# Autodesk Inventor assembly: outside_sleds_MIR
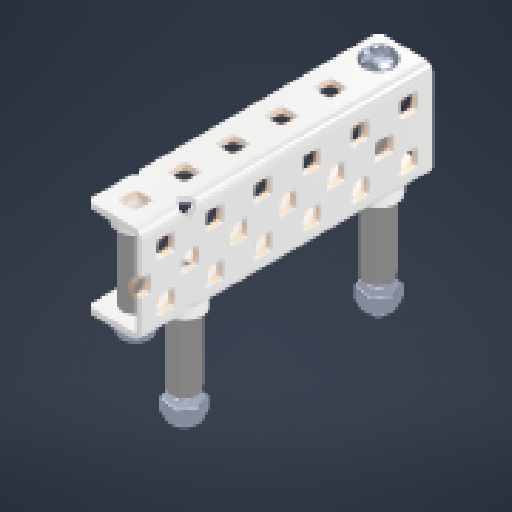
[picture p0: Inventor's stored thumbnail of the model, 512x512]
Saved by Autodesk Inventor 2023 (Build 270158000, 158)
## iProperties
Created: 2023-08-07
Part Number: outside_sleds_MIR
Document SubType Name: Assembly
Designer: srbel
Author: srbel
## Documents named in this file (10)
- C:\CAD\OverUnderCAD\Drive\outside_sleds_MIR.iam
- C:\CAD\OverUnderCAD\VEX-CAD-Inventor-1.4.0\Structure\C Channel\Aluminum 1x2x1\Alu C 1x2x1x6_MIR.ipt
- C:\CAD\OverUnderCAD\VEX-CAD-Inventor-1.4.0\Motion\Spacers\Spacer Nylon .313 OD\NSpacer .313 OD x .125.ipt
- C:\CAD\OverUnderCAD\VEX-CAD-Inventor-1.4.0\Motion\Spacers\Spacer Nylon .313 OD.ipt
- C:\CAD\OverUnderCAD\VEX-CAD-Inventor-1.4.0\Structure\Standoff\Standoff .75.ipt
- C:\CAD\OverUnderCAD\VEX-CAD-Inventor-1.4.0\Structure\Standoff.ipt
- C:\CAD\OverUnderCAD\VEX-CAD-Inventor-1.4.0\Structure\Hardware\Screw Steel - Star\SScrew Star Threaded 2.250.ipt
- C:\CAD\OverUnderCAD\VEX-CAD-Inventor-1.4.0\Structure\Hardware\Screw Steel - Star.ipt
- C:\CAD\OverUnderCAD\VEX-CAD-Inventor-1.4.0\Structure\Hardware\Screw Steel - Star\SScrew Star Threaded 1.250.ipt
- C:\CAD\OverUnderCAD\VEX-CAD-Inventor-1.4.0\Structure\Hardware\Nut Thin Nylock.ipt
## Components (14 placed, 6 different names)
1. Alu C 1x2x1x6_MIR:1 — Insert:1, Insert:3, Insert:6, Insert:7, Insert:9, Insert:11, Insert:12
2. NSpacer .313 OD x .125:1 — Insert:1, Insert:2
3. Standoff .75:1 — Insert:2
4. NSpacer .313 OD x .125:2 — Insert:3, Insert:4
5. Standoff .75:2 — Insert:4
6. NSpacer .313 OD x .125:3 — Insert:6, Insert:5
7. Standoff .75:3 — Insert:5, Insert:14
8. NSpacer .313 OD x .125:4 — Insert:7, Insert:8
9. Standoff .75:4 — Insert:8, Insert:13
10. SScrew Star Threaded 2.250:1 — Insert:9
11. SScrew Star Threaded 1.250:3 — Insert:11
12. Nut Thin Nylock:1 — Insert:12
13. Nut Thin Nylock:2 — Insert:13
14. Nut Thin Nylock:3 — Insert:14
## Relationships (13: Insert 13)
- Insert:1: Alu C 1x2x1x6_MIR:1 ↔ NSpacer .313 OD x .125:1
- Insert:2: NSpacer .313 OD x .125:1 ↔ Standoff .75:1
- Insert:3: Alu C 1x2x1x6_MIR:1 ↔ NSpacer .313 OD x .125:2
- Insert:4: NSpacer .313 OD x .125:2 ↔ Standoff .75:2
- Insert:6 (1.5875 mm): Alu C 1x2x1x6_MIR:1 ↔ NSpacer .313 OD x .125:3
- Insert:5: NSpacer .313 OD x .125:3 ↔ Standoff .75:3
- Insert:7 (1.5875 mm): Alu C 1x2x1x6_MIR:1 ↔ NSpacer .313 OD x .125:4
- Insert:8: NSpacer .313 OD x .125:4 ↔ Standoff .75:4
- Insert:9: Alu C 1x2x1x6_MIR:1 ↔ SScrew Star Threaded 2.250:1
- Insert:11: Alu C 1x2x1x6_MIR:1 ↔ SScrew Star Threaded 1.250:3
- Insert:12: Alu C 1x2x1x6_MIR:1 ↔ Nut Thin Nylock:1
- Insert:13 (1.5875 mm): Standoff .75:4 ↔ Nut Thin Nylock:2
- Insert:14 (1.5875 mm): Standoff .75:3 ↔ Nut Thin Nylock:3
